# Autodesk Inventor assembly: 200-60-DIFFERENTIAL-CONNECTOR-01
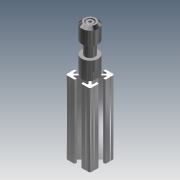
[picture p0: Inventor's stored thumbnail of the model, 180x180]
Saved by Autodesk Inventor 2018.2 (Build 222227000, 227)
## iProperties
Manager: feesmrt
Company: FRANC0R
Created: 2017-12-18
Part Number: 200-60-DIFFERENTIAL-CONNECTOR-01
Document SubType Name: Assembly
Designer: feesmrt
Project: Rescue Robot
Cost Center: -
Description: Differential Connector ASM
Engineer: feesmrt
Authority: feesmrt
Stock Number: 200-60-DIFFERENTIAL-CONNECTOR-01
Author: feesmrt
Title: Differential Connector ASM
Subject: Recue Robot
Revision Number: 1
## Documents named in this file (5)
- D:\Programmierung\FRANC0R\CAD\02-Rocker-Bogie-Robot\200-ROCKER-BOGIE\200-60-DIFFERENTIAL\200-60-DIFFERENTIAL-CONNECTOR-01.iam
- D:\Programmierung\FRANC0R\CAD\02-Rocker-Bogie-Robot\200-ROCKER-BOGIE\200-60-DIFFERENTIAL\200-60-DIFFERENTIAL-CONNECTOR-02.ipt
- D:\Programmierung\FRANC0R\CAD\02-Rocker-Bogie-Robot\200-ROCKER-BOGIE\200-60-DIFFERENTIAL\200-60-DIFFERENTIAL-CONNECTOR-03.ipt
- D:\Programmierung\FRANC0R\CAD\02-Rocker-Bogie-Robot\900-COMPONENTS\900-40-SCREWS\900-40-SCREWS-DIN7984_M5x12.ipt
- D:\Programmierung\FRANC0R\CAD\02-Rocker-Bogie-Robot\200-ROCKER-BOGIE\200-60-DIFFERENTIAL\200-60-DIFFERENTIAL-PROFILE-01.ipt
## Components (4 placed, 4 different names)
1. 200-60-DIFFERENTIAL-CONNECTOR-02:1 — Passend:1, Passend:2, Passend:5, Passend:6
2. 200-60-DIFFERENTIAL-CONNECTOR-03:1 — Passend:1, Passend:2, Passend:3, Passend:4
3. 900-40-SCREWS-DIN7984_M5x12:1 — Passend:3, Passend:4
4. 200-60-DIFFERENTIAL-PROFILE-01:1 — Passend:5, Passend:6, Passend:7
## Relationships (7: Mate 7)
- Passend:1 [Mate]: 200-60-DIFFERENTIAL-CONNECTOR-02:1 ↔ 200-60-DIFFERENTIAL-CONNECTOR-03:1
- Passend:2 [Mate]: 200-60-DIFFERENTIAL-CONNECTOR-02:1 ↔ 200-60-DIFFERENTIAL-CONNECTOR-03:1
- Passend:3 [Mate]: 200-60-DIFFERENTIAL-CONNECTOR-03:1 ↔ 900-40-SCREWS-DIN7984_M5x12:1
- Passend:4 [Mate]: 200-60-DIFFERENTIAL-CONNECTOR-03:1 ↔ 900-40-SCREWS-DIN7984_M5x12:1
- Passend:5 [Mate]: 200-60-DIFFERENTIAL-CONNECTOR-02:1 ↔ 200-60-DIFFERENTIAL-PROFILE-01:1
- Passend:6 [Mate]: 200-60-DIFFERENTIAL-CONNECTOR-02:1 ↔ 200-60-DIFFERENTIAL-PROFILE-01:1
- Passend:7 [Mate]: 200-60-DIFFERENTIAL-PROFILE-01:1
